# Autodesk Inventor assembly: Expansion_Module_Assembly
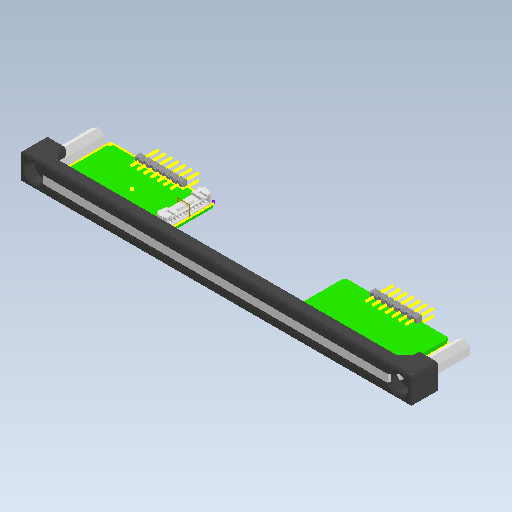
[picture p0: Inventor's stored thumbnail of the model, 512x512]
Saved by Autodesk Inventor 2021 (Build 250183000, 183)
## iProperties
Created: 2020-07-14
Part Number: Expansion_Module_Assembly
Document SubType Name: Assembly
Designer: CASE-SMALL2
Author: CASE-SMALL2
## Documents named in this file (5)
- C:\Users\Viktor\Google Drive\Unicorn 2020\CAD_V2\PCB_Assemblies\Expansion_Module_Assembly.iam
- C:\Users\Viktor\Google Drive\Unicorn 2020\CAD_V2\PCB_Assemblies\Other\ModuleBracket.ipt
- C:\Users\Viktor\Google Drive\Unicorn 2020\CAD_V2\PCB_Assemblies\Standsoffs\M2.5x20mm_Standoff_ 970200144.ipt
- C:\Users\Viktor\Google Drive\Unicorn 2020\CAD_V2\PCB_Assemblies\Expansion_Module_PCB_Assembly.iam
- C:\Users\Viktor\Google Drive\Unicorn 2020\CAD_V2\PCB_Assemblies\Other\ModuleBracket_Slot.ipt
## Components (6 placed, 4 different names)
1. ModuleBracket:1 — Rigid:1, Rigid:2, Flush:3, Mate:1, Rigid:3
2. M2.5x20mm_Standoff_ 970200144:1 — Rigid:1, Flush:4, Flush:5
3. M2.5x20mm_Standoff_ 970200144:2 — Rigid:2, Flush:1, Flush:2
4. Expansion_Module_PCB_Assembly:1 [sub-assembly] — Flush:1, Flush:2, Flush:3
5. Expansion_Module_PCB_Assembly:2 [sub-assembly] — Flush:4, Flush:5, Mate:1
6. ModuleBracket_Slot:1 — Rigid:3
## Relationships (9: Flush 5, WeldJoint 3, Mate 1)
- Rigid:1 [WeldJoint]: ModuleBracket:1 ↔ M2.5x20mm_Standoff_ 970200144:1
- Rigid:2 [WeldJoint]: ModuleBracket:1 ↔ M2.5x20mm_Standoff_ 970200144:2
- Flush:1: M2.5x20mm_Standoff_ 970200144:2 ↔ Expansion_Module_PCB_Assembly:1
- Flush:2 (7.5 mm): M2.5x20mm_Standoff_ 970200144:2 ↔ Expansion_Module_PCB_Assembly:1
- Flush:3: ModuleBracket:1 ↔ Expansion_Module_PCB_Assembly:1
- Flush:4 (7.5 mm): M2.5x20mm_Standoff_ 970200144:1 ↔ Expansion_Module_PCB_Assembly:2
- Flush:5: M2.5x20mm_Standoff_ 970200144:1 ↔ Expansion_Module_PCB_Assembly:2
- Mate:1: ModuleBracket:1 ↔ Expansion_Module_PCB_Assembly:2
- Rigid:3 [WeldJoint]: ModuleBracket:1 ↔ ModuleBracket_Slot:1
